# Autodesk Inventor assembly: B Drive
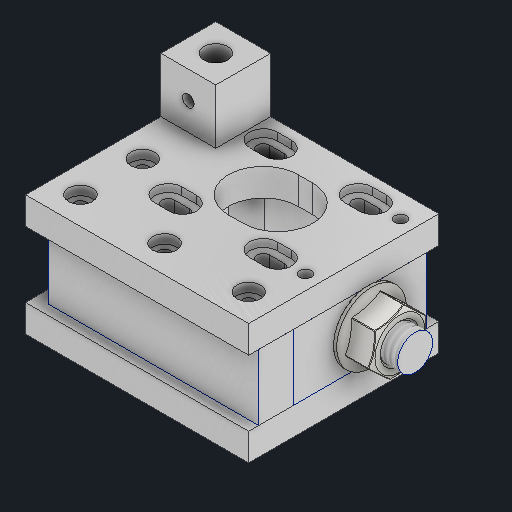
[picture p0: Inventor's stored thumbnail of the model, 512x512]
Saved by Autodesk Inventor 2025.1 (Build 291241020, 241B)
## iProperties
Created: 2025-04-19
Part Number: B Drive
Document SubType Name: Assembly
Designer: Joshua Eah
Mass: 215.49 g
Surface Area: 286.778 cm^2
Volume: 59.2862 cm^3
Density: 3.63475 g/cm^3
Author: Joshua Eah
## Documents named in this file (9)
- C:\Users\Joshua Eah\Documents\Voron 0.2\CAD\Machined Parts\AB Drives\B Drive\B Drive Assembly.iam
- C:\Users\Joshua Eah\Documents\Voron 0.2\CAD\Machined Parts\AB Drives\B Drive\B Drive Frame Lower.ipt
- C:\Users\Joshua Eah\Documents\Voron 0.2\CAD\Machined Parts\AB Drives\B Drive\B Drive Frame Upper.ipt
- C:\Users\Joshua Eah\Documents\Voron 0.2\CAD\Machined Parts\AB Drives\Drive Tensioner Rod\Tensioner Rod.ipt
- C:\Users\Joshua Eah\Documents\Voron 0.2\CAD\Machined Parts\AB Drives\Drive Frame Bearing Plate\Drive Frame Tension Bearing Plate.ipt
- C:\Users\Joshua Eah\Documents\Voron 0.2\CAD\Machined Parts\AB Drives\Drive Tensioner\Drive Tensioner.ipt
- C:\Users\Joshua Eah\Documents\Voron 0.2\CAD\Machined Parts\AB Drives\3_8_16_Nut.ipt
- C:\Users\Joshua Eah\Documents\Voron 0.2\CAD\Machined Parts\AB Drives\Drive Frame Spacer\Drive Frame Spacing Block.ipt
- C:\Users\Joshua Eah\Documents\Voron 0.2\CAD\Machined Parts\Spacers\Spacer.ipt
## Components (8 placed, 8 different names)
1. B Drive Frame Lower:1 — Rigid:4, Rigid:5, Slider:1, Mate:1
2. B Drive Frame Upper:1 — Rigid:6
3. Drive Tensioner:1 — Rigid:1, Slider:1
4. Tensioner Rod:1 — Rigid:1, Cylindrical:1
5. Drive Frame Tension Bearing Plate:1 — Rigid:4
6. 3_8_16_Nut:1 — Cylindrical:1
7. Drive Frame Spacing Block:1 — Rigid:5, Rigid:6
8. Spacer:1 — Mate:1
## Relationships (7: WeldJoint 4, CylindricalJoint 1, TranslationJoint 1, Mate 1)
- Rigid:1 [WeldJoint]: Drive Tensioner:1 ↔ Tensioner Rod:1
- Cylindrical:1: Tensioner Rod:1 ↔ 3_8_16_Nut:1
- Rigid:4 [WeldJoint]: B Drive Frame Lower:1 ↔ Drive Frame Tension Bearing Plate:1
- Rigid:5 [WeldJoint]: B Drive Frame Lower:1 ↔ Drive Frame Spacing Block:1
- Slider:1 [TranslationJoint]: B Drive Frame Lower:1 ↔ Drive Tensioner:1
- Rigid:6 [WeldJoint]: B Drive Frame Upper:1 ↔ Drive Frame Spacing Block:1
- Mate:1: B Drive Frame Lower:1 ↔ Spacer:1
